# Autodesk Inventor assembly: electronics
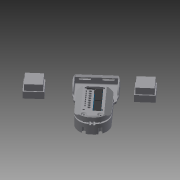
[picture p0: Inventor's stored thumbnail of the model, 180x180]
Saved by Autodesk Inventor 2014 (Build 180170000, 170)
## iProperties
Created: 2014-05-24
Part Number: electronics
Document SubType Name: Assembly
Designer: brent
Author: brent
## Documents named in this file (6)
- C:\Users\brent\Documents\electric-longboard\brent\electronics.iam
- C:\Users\brent\Documents\electric-longboard\brent\electronicsbox_top.ipt
- C:\Users\brent\Documents\electric-longboard\brent\electronicsbox_lid.ipt
- C:\Users\brent\Documents\electric-longboard\brent\tm1638module.ipt
- C:\Users\brent\Documents\electric-longboard\brent\hobbyking150acaresc.ipt
- C:\Users\brent\Documents\electric-longboard\brent\electronicsbox_button.ipt
## Components (13 placed, 5 different names)
1. electronicsbox_top:1 — Mate:4, Mate:5, Mate:6, Mate:7, Mate:8, Mate:9, Mate:18
2. electronicsbox_lid:1 — Mate:1, Mate:2, Mate:3, Mate:4, Mate:5, Mate:10, Mate:11, Mate:12, Mate:13, Mate:14, Mate:15, Mate:16, Mate:17, Flush:8, Mate:18
3. tm1638module:1 — Mate:1, Mate:2, Mate:3
4. hobbyking150acaresc:1 — Mate:6, Mate:8
5. hobbyking150acaresc:2 — Mate:7, Mate:9
6. electronicsbox_button:1 — Mate:10, Flush:1, Flush:2, Flush:3, Flush:4, Flush:5, Flush:6, Flush:7, Flush:8
7. electronicsbox_button:2 — Mate:11, Flush:1
8. electronicsbox_button:3 — Mate:14, Flush:4
9. electronicsbox_button:4 — Mate:15, Flush:5
10. electronicsbox_button:5 — Mate:13, Flush:3
11. electronicsbox_button:6 — Mate:12, Flush:2
12. electronicsbox_button:7 — Mate:16, Flush:6
13. electronicsbox_button:8 — Mate:17, Flush:7
## Relationships (26: Mate 18, Flush 8)
- Mate:1: electronicsbox_lid:1 ↔ tm1638module:1
- Mate:2: electronicsbox_lid:1 ↔ tm1638module:1
- Mate:3: electronicsbox_lid:1 ↔ tm1638module:1
- Mate:4: electronicsbox_top:1 ↔ electronicsbox_lid:1
- Mate:5: electronicsbox_top:1 ↔ electronicsbox_lid:1
- Mate:6: electronicsbox_top:1 ↔ hobbyking150acaresc:1
- Mate:7: electronicsbox_top:1 ↔ hobbyking150acaresc:2
- Mate:8 (3.81 mm): electronicsbox_top:1 ↔ hobbyking150acaresc:1
- Mate:9 (3.81 mm): electronicsbox_top:1 ↔ hobbyking150acaresc:2
- Mate:10: electronicsbox_lid:1 ↔ electronicsbox_button:1
- Mate:11: electronicsbox_lid:1 ↔ electronicsbox_button:2
- Mate:12: electronicsbox_lid:1 ↔ electronicsbox_button:6
- Mate:13: electronicsbox_lid:1 ↔ electronicsbox_button:5
- Mate:14: electronicsbox_lid:1 ↔ electronicsbox_button:3
- Mate:15: electronicsbox_lid:1 ↔ electronicsbox_button:4
- Mate:16: electronicsbox_lid:1 ↔ electronicsbox_button:7
- Mate:17: electronicsbox_lid:1 ↔ electronicsbox_button:8
- Flush:1: electronicsbox_button:1 ↔ electronicsbox_button:2
- Flush:2: electronicsbox_button:1 ↔ electronicsbox_button:6
- Flush:3: electronicsbox_button:1 ↔ electronicsbox_button:5
- Flush:4: electronicsbox_button:1 ↔ electronicsbox_button:3
- Flush:5: electronicsbox_button:1 ↔ electronicsbox_button:4
- Flush:6: electronicsbox_button:1 ↔ electronicsbox_button:7
- Flush:7: electronicsbox_button:1 ↔ electronicsbox_button:8
- Flush:8: electronicsbox_lid:1 ↔ electronicsbox_button:1
- Mate:18 (1.27 mm): electronicsbox_top:1 ↔ electronicsbox_lid:1
